# Autodesk Inventor assembly: group_3_robot
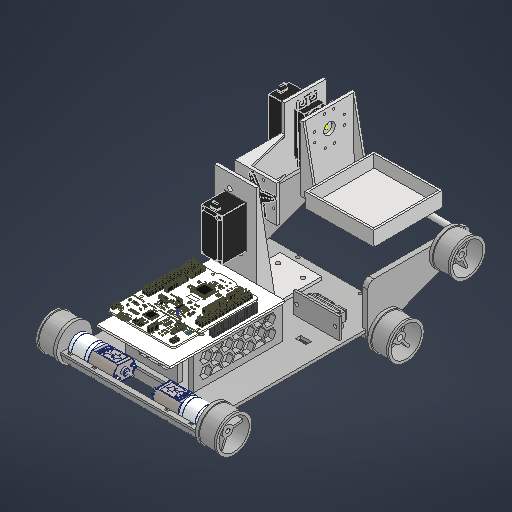
[picture p0: Inventor's stored thumbnail of the model, 512x512]
Saved by Autodesk Inventor 2026 (Build 300175000, 175)
## iProperties
Created: 2025-07-07
Part Number: group_3_robot
Document SubType Name: Assembly
Designer: user
Author: user
## Documents named in this file (16)
- C:\Users\user\Mbed Programs\System_Engineering_of_pes_board\temp\Cad_files\Chassis\group_3_robot.iam
- C:\Users\user\Mbed Programs\System_Engineering_of_pes_board\temp\Cad_files\Chassis\Robot_Chassis_Bottom.ipt
- C:\Users\user\Mbed Programs\System_Engineering_of_pes_board\temp\Cad_files\Chassis\BatteryPack v6.ipt
- C:\Users\user\Mbed Programs\System_Engineering_of_pes_board\temp\Cad_files\Gimble\pan_base_holder_first_v1.ipt
- C:\Users\user\Mbed Programs\System_Engineering_of_pes_board\temp\Cad_files\Chassis\Assembly_Patrs_Robot\Assembly_Patrs_Robot\pes-board v1.ipt
- C:\Users\user\Mbed Programs\System_Engineering_of_pes_board\temp\Cad_files\Chassis\Assembly_Patrs_Robot\Assembly_Patrs_Robot\STM32NUCLEO v1.ipt
- C:\Users\user\Mbed Programs\System_Engineering_of_pes_board\temp\Cad_files\Chassis\20d-metal-gearmotor-100-125-156-195-with-extended-motor-shaft v1.ipt
- C:\Users\user\Mbed Programs\System_Engineering_of_pes_board\temp\Cad_files\Chassis\Assembly_Patrs_Robot\Rad v2.ipt
- C:\Users\user\Mbed Programs\System_Engineering_of_pes_board\temp\Cad_files\Chassis\Assembly_Patrs_Robot\rod_connecting.ipt
- C:\Users\user\Mbed Programs\System_Engineering_of_pes_board\temp\Cad_files\Chassis\Assembly_Patrs_Robot\Rad v3.ipt
- C:\Users\user\Mbed Programs\System_Engineering_of_pes_board\temp\Cad_files\Chassis\IR_sensor v1\IR_sensor v1\IR_sensor v1.ipt
- C:\Users\user\Mbed Programs\System_Engineering_of_pes_board\temp\Cad_files\Gimble\Servo Futaba S3003 v6\Servo Futaba S3003 v6\Part4.ipt
- C:\Users\user\Mbed Programs\System_Engineering_of_pes_board\temp\Cad_files\Gimble\Servo Futaba S3003 v6\Servo Futaba S3003 v6\Aspa_creu_Axix holder_v2_one_flap.ipt
- C:\Users\user\Mbed Programs\System_Engineering_of_pes_board\temp\Cad_files\Gimble\pan_base_holder_second.ipt
- C:\Users\user\Mbed Programs\System_Engineering_of_pes_board\temp\Cad_files\Gimble\pan_base_holder_third.ipt
- C:\Users\user\Mbed Programs\System_Engineering_of_pes_board\temp\Cad_files\Chassis\Differential_drive_wheel.ipt
## Components (24 placed, 15 different names)
1. Robot_Chassis_Bottom:1 — Mate:1, Mate:2, Mate:3, Mate:4, Mate:12, Mate:14, Mate:18, Flush:5, Flush:6, Mate:23, Mate:24, Mate:25, Mate:42, Mate:46, Mate:47, Mate:48, Mate:49, Flush:11, Mate:50, Mate:51, Flush:12, Mate:52
2. BatteryPack v6:1 — Mate:1, Mate:2, Mate:3, Mate:7, Mate:9
3. pan_base_holder_first_v1:1 — Mate:4, Mate:27, Mate:28, Mate:41, Mate:47, Mate:48
4. pes-board v1:1 — Mate:7, Mate:9, Mate:10, Flush:1, Flush:2
5. STM32NUCLEO v1:1 — Mate:10, Flush:1, Flush:2
6. 20d-metal-gearmotor-100-125-156-195-with-extended-motor-shaft v1:1 — Mate:14, Mate:16, Flush:4, Mate:45, Mate:46
7. 20d-metal-gearmotor-100-125-156-195-with-extended-motor-shaft v1:2 — Mate:12, Mate:15, Flush:3, Mate:45
8. Rad v2:1 — Mate:15, Flush:3
9. Rad v2:2 — Mate:16, Flush:4
10. rod_connecting:1 — Flush:5, Flush:7, Flush:10, Mate:42, Mate:43
11. rod_connecting:2 — Mate:18, Flush:6, Mate:20, Mate:21, Flush:8, Flush:9
12. Rad v3:1 — Flush:7
13. Rad v3:2 — Mate:21, Flush:9
14. Rad v3:3 — Mate:20, Flush:8
15. Rad v3:4 — Flush:10, Mate:43
16. IR_sensor v1:1 — Mate:23, Mate:24, Mate:25
17. Part4:1 — Mate:27, Mate:28, Mate:29, Mate:30, Mate:41
18. Aspa_creu_Axix holder_v2_one_flap:1 — Mate:29, Mate:30, Mate:31, Mate:32
19. pan_base_holder_second:1 — Mate:31, Mate:32, Mate:33, Mate:34, Mate:35
20. Part4:2 — Mate:33, Mate:34, Mate:35, Mate:36, Mate:37
21. Aspa_creu_Axix holder_v2_one_flap:2 — Mate:36, Mate:37, Mate:38, Mate:39
22. pan_base_holder_third:1 — Mate:38, Mate:39
23. Differential_drive_wheel:1 — Mate:49, Flush:11, Mate:50
24. Differential_drive_wheel:2 — Mate:51, Flush:12, Mate:52
## Relationships (53: Mate 41, Flush 12)
- Mate:1: Robot_Chassis_Bottom:1 ↔ BatteryPack v6:1
- Mate:2: Robot_Chassis_Bottom:1 ↔ BatteryPack v6:1
- Mate:3: Robot_Chassis_Bottom:1 ↔ BatteryPack v6:1
- Mate:4: Robot_Chassis_Bottom:1 ↔ pan_base_holder_first_v1:1
- Mate:7: BatteryPack v6:1 ↔ pes-board v1:1
- Mate:9: BatteryPack v6:1 ↔ pes-board v1:1
- Mate:10 (9 mm): pes-board v1:1 ↔ STM32NUCLEO v1:1
- Flush:1 (3 mm): pes-board v1:1 ↔ STM32NUCLEO v1:1
- Flush:2 (19 mm): pes-board v1:1 ↔ STM32NUCLEO v1:1
- Mate:12: Robot_Chassis_Bottom:1 ↔ 20d-metal-gearmotor-100-125-156-195-with-extended-motor-shaft v1:2
- Mate:14: Robot_Chassis_Bottom:1 ↔ 20d-metal-gearmotor-100-125-156-195-with-extended-motor-shaft v1:1
- Mate:15: 20d-metal-gearmotor-100-125-156-195-with-extended-motor-shaft v1:2 ↔ Rad v2:1
- Mate:16: 20d-metal-gearmotor-100-125-156-195-with-extended-motor-shaft v1:1 ↔ Rad v2:2
- Flush:3: 20d-metal-gearmotor-100-125-156-195-with-extended-motor-shaft v1:2 ↔ Rad v2:1
- Flush:4: 20d-metal-gearmotor-100-125-156-195-with-extended-motor-shaft v1:1 ↔ Rad v2:2
- Mate:18: Robot_Chassis_Bottom:1 ↔ rod_connecting:2
- Flush:5 (-16 mm): Robot_Chassis_Bottom:1 ↔ rod_connecting:1
- Flush:6 (-16 mm): Robot_Chassis_Bottom:1 ↔ rod_connecting:2
- Flush:7: rod_connecting:1 ↔ Rad v3:1
- Mate:20: rod_connecting:2 ↔ Rad v3:3
- Mate:21: rod_connecting:2 ↔ Rad v3:2
- Flush:8: rod_connecting:2 ↔ Rad v3:3
- Flush:9: rod_connecting:2 ↔ Rad v3:2
- Flush:10: rod_connecting:1 ↔ Rad v3:4
- Mate:23: Robot_Chassis_Bottom:1 ↔ IR_sensor v1:1
- Mate:24: Robot_Chassis_Bottom:1 ↔ IR_sensor v1:1
- Mate:25: Robot_Chassis_Bottom:1 ↔ IR_sensor v1:1
- Mate:27 (0.25 mm): pan_base_holder_first_v1:1 ↔ Part4:1
- Mate:28: pan_base_holder_first_v1:1 ↔ Part4:1
- Mate:29: Part4:1 ↔ Aspa_creu_Axix holder_v2_one_flap:1
- Mate:30: Part4:1 ↔ Aspa_creu_Axix holder_v2_one_flap:1
- Mate:31: Aspa_creu_Axix holder_v2_one_flap:1 ↔ pan_base_holder_second:1
- Mate:32: Aspa_creu_Axix holder_v2_one_flap:1 ↔ pan_base_holder_second:1
- Mate:33 (0.5 mm): pan_base_holder_second:1 ↔ Part4:2
- Mate:34 (0.25 mm): pan_base_holder_second:1 ↔ Part4:2
- Mate:35: pan_base_holder_second:1 ↔ Part4:2
- Mate:36: Part4:2 ↔ Aspa_creu_Axix holder_v2_one_flap:2
- Mate:37: Part4:2 ↔ Aspa_creu_Axix holder_v2_one_flap:2
- Mate:38: Aspa_creu_Axix holder_v2_one_flap:2 ↔ pan_base_holder_third:1
- Mate:39: Aspa_creu_Axix holder_v2_one_flap:2 ↔ pan_base_holder_third:1
- Mate:41 (0.5 mm): pan_base_holder_first_v1:1 ↔ Part4:1
- Mate:42: Robot_Chassis_Bottom:1 ↔ rod_connecting:1
- Mate:43: rod_connecting:1 ↔ Rad v3:4
- Mate:45: 20d-metal-gearmotor-100-125-156-195-with-extended-motor-shaft v1:1 ↔ 20d-metal-gearmotor-100-125-156-195-with-extended-motor-shaft v1:2
- Mate:46: Robot_Chassis_Bottom:1 ↔ 20d-metal-gearmotor-100-125-156-195-with-extended-motor-shaft v1:1
- Mate:47: Robot_Chassis_Bottom:1 ↔ pan_base_holder_first_v1:1
- Mate:48: Robot_Chassis_Bottom:1 ↔ pan_base_holder_first_v1:1
- Mate:49: Robot_Chassis_Bottom:1 ↔ Differential_drive_wheel:1
- Flush:11: Robot_Chassis_Bottom:1 ↔ Differential_drive_wheel:1
- Mate:50: Robot_Chassis_Bottom:1 ↔ Differential_drive_wheel:1
- Mate:51: Robot_Chassis_Bottom:1 ↔ Differential_drive_wheel:2
- Flush:12: Robot_Chassis_Bottom:1 ↔ Differential_drive_wheel:2
- Mate:52: Robot_Chassis_Bottom:1 ↔ Differential_drive_wheel:2
